# Autodesk Inventor assembly: Ra-Manager_Montagem_Plugs
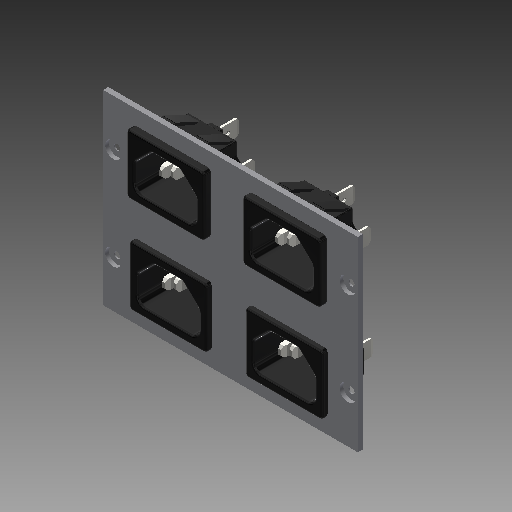
[picture p0: Inventor's stored thumbnail of the model, 512x512]
Saved by Autodesk Inventor 2019.4 (Build 234330000, 330)
## iProperties
Created: 2020-03-24
Part Number: Ra-Manager_Montagem_Plugs
Material: Genérico
Document SubType Name: Assembly
Designer: caiom
Author: caiom
## Documents named in this file (3)
- C:\Users\caiom\Desktop\Ra-Manager_Mecanica\Ra-Manager_Montagem_Plugs.iam
- C:\Users\caiom\Desktop\Ra-Manager_Mecanica\Ra-Manager_Painel-Placas_Tras_Plugs.ipt
- C:\Users\caiom\Desktop\Ra-Manager_Mecanica\IEC Plug\AC_power_jack.ipt
## Components (5 placed, 2 different names)
1. Ra-Manager_Painel-Placas_Tras_Plugs:1 — Coincidência:1, Alinhamento:1, Alinhamento:2, Coincidência:2, Alinhamento:3, Alinhamento:4, Alinhamento:5, Alinhamento:6, Alinhamento:7, Alinhamento:8
2. AC_power_jack:1 — Coincidência:1, Alinhamento:1, Alinhamento:2
3. AC_power_jack:2 — Coincidência:2, Alinhamento:3, Alinhamento:4
4. AC_power_jack:3 — Alinhamento:5, Alinhamento:6
5. AC_power_jack:4 — Alinhamento:7, Alinhamento:8
## Relationships (10: Flush 8, Mate 2)
- Coincidência:1 [Mate]: Ra-Manager_Painel-Placas_Tras_Plugs:1 ↔ AC_power_jack:1
- Alinhamento:1 [Flush] (5.5 mm): Ra-Manager_Painel-Placas_Tras_Plugs:1 ↔ AC_power_jack:1
- Alinhamento:2 [Flush] (12 mm): Ra-Manager_Painel-Placas_Tras_Plugs:1 ↔ AC_power_jack:1
- Coincidência:2 [Mate]: Ra-Manager_Painel-Placas_Tras_Plugs:1 ↔ AC_power_jack:2
- Alinhamento:3 [Flush] (5.5 mm): Ra-Manager_Painel-Placas_Tras_Plugs:1 ↔ AC_power_jack:2
- Alinhamento:4 [Flush] (12 mm): Ra-Manager_Painel-Placas_Tras_Plugs:1 ↔ AC_power_jack:2
- Alinhamento:5 [Flush] (5.5 mm): Ra-Manager_Painel-Placas_Tras_Plugs:1 ↔ AC_power_jack:3
- Alinhamento:6 [Flush] (12 mm): Ra-Manager_Painel-Placas_Tras_Plugs:1 ↔ AC_power_jack:3
- Alinhamento:7 [Flush] (5.5 mm): Ra-Manager_Painel-Placas_Tras_Plugs:1 ↔ AC_power_jack:4
- Alinhamento:8 [Flush] (12 mm): Ra-Manager_Painel-Placas_Tras_Plugs:1 ↔ AC_power_jack:4
